# Autodesk Inventor assembly: Splitter Assembly
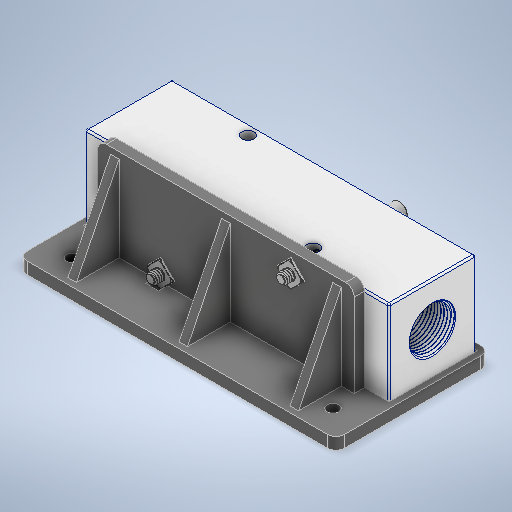
[picture p0: Inventor's stored thumbnail of the model, 512x512]
Saved by Autodesk Inventor 2025 (Build 290162000, 162)
## iProperties
Created: 2025-03-12
Part Number: Splitter Assembly
Document SubType Name: Assembly
Designer: Caleb Fangmeier
Author: Caleb Fangmeier
## Documents named in this file (5)
- C:\Users\cfang\Desktop\nebraska-silicon-lab\Hardware\General Gantry\Splitter Mount\Splitter Assembly.iam
- C:\Users\cfang\Desktop\nebraska-silicon-lab\Hardware\General Gantry\Splitter Mount\5469K249_Anodized Aluminum Right-Angle Flow Manifold\5469K249_Anodized Aluminum Right-Angle Flow Manifold.ipt
- C:\Users\cfang\Desktop\nebraska-silicon-lab\Hardware\General Gantry\Splitter Mount\Splitter Mount.ipt
- C:\Users\cfang\Desktop\nebraska-silicon-lab\Hardware\General Gantry\Splitter Mount\94855A247_Low-Strength Steel Square Nut\94855A247_Low-Strength Steel Square Nut.ipt
- C:\Users\cfang\Desktop\nebraska-silicon-lab\Hardware\General Gantry\Splitter Mount\90128A255_Zinc-Plated Alloy Steel Socket Head Screw\90128A255_Zinc-Plated Alloy Steel Socket Head Screw.ipt
## Components (6 placed, 4 different names)
1. 5469K249_Anodized Aluminum Right-Angle Flow Manifold:1 — Mate:1, Mate:2, Mate:3, Insert:1, Insert:2
2. Splitter Mount:1 — Mate:1, Mate:2, Mate:3, Mate:4, Angle:1, Mate:5, Angle:2
3. 94855A247_Low-Strength Steel Square Nut:1 — Mate:4, Angle:1
4. 94855A247_Low-Strength Steel Square Nut:2 — Mate:5, Angle:2
5. 90128A255_Zinc-Plated Alloy Steel Socket Head Screw:1 — Insert:1
6. 90128A255_Zinc-Plated Alloy Steel Socket Head Screw:2 — Insert:2
## Relationships (9: Mate 5, Angle 2, Insert 2)
- Mate:1: 5469K249_Anodized Aluminum Right-Angle Flow Manifold:1 ↔ Splitter Mount:1
- Mate:2 (0.5 mm): 5469K249_Anodized Aluminum Right-Angle Flow Manifold:1 ↔ Splitter Mount:1
- Mate:3 (0.5 mm): 5469K249_Anodized Aluminum Right-Angle Flow Manifold:1 ↔ Splitter Mount:1
- Mate:4: Splitter Mount:1 ↔ 94855A247_Low-Strength Steel Square Nut:1
- Angle:1 (0 deg): Splitter Mount:1 ↔ 94855A247_Low-Strength Steel Square Nut:1
- Mate:5: Splitter Mount:1 ↔ 94855A247_Low-Strength Steel Square Nut:2
- Angle:2 (0 deg): Splitter Mount:1 ↔ 94855A247_Low-Strength Steel Square Nut:2
- Insert:1: 5469K249_Anodized Aluminum Right-Angle Flow Manifold:1 ↔ 90128A255_Zinc-Plated Alloy Steel Socket Head Screw:1
- Insert:2: 5469K249_Anodized Aluminum Right-Angle Flow Manifold:1 ↔ 90128A255_Zinc-Plated Alloy Steel Socket Head Screw:2
